# Autodesk Inventor assembly: Dog Feeder _Caja
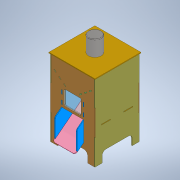
[picture p0: Inventor's stored thumbnail of the model, 180x180]
Saved by Autodesk Inventor 2020.1 (Build 241239000, 239)
## iProperties
Created: 2019-12-08
Part Number: Dog Feeder _Caja
Document SubType Name: Assembly
Designer: Daniel
Author: Daniel
## Documents named in this file (18)
- F:\Proyectos\Dog Feeder\Solido\Version Caja\Dog Feeder _Caja.iam
- F:\Proyectos\Dog Feeder\Solido\Ensamble Inicial\Ensamble inicial_ Dog Feeder.iam
- F:\Proyectos\Dog Feeder\Solido\Version Caja\Soporte_Rodamientos.ipt
- F:\Proyectos\Dog Feeder\Solido\Version Caja\Soporte2_Rodamientos.ipt
- F:\Proyectos\Dog Feeder\Solido\Rodamiento\6202-Z.iam
- F:\Proyectos\Dog Feeder\Solido\Version Caja\Rampa.ipt
- F:\Proyectos\Dog Feeder\Solido\Version Caja\Suelo.ipt
- F:\Proyectos\Dog Feeder\Solido\Version Caja\Pared_Lateral.ipt
- F:\Proyectos\Dog Feeder\Solido\Version Caja\Pared_Trasera.ipt
- F:\Proyectos\Dog Feeder\Solido\Version Caja\Tolva_Largo.ipt
- F:\Proyectos\Dog Feeder\Solido\Version Caja\Tolva_Corto.ipt
- F:\Proyectos\Dog Feeder\Solido\Version Caja\Pared_Frontal.ipt
- F:\Proyectos\Dog Feeder\Solido\Version Caja\Ventana.ipt
- F:\Proyectos\Dog Feeder\Solido\Circuito Electrico\Circuito_Electrico.iam
- F:\Proyectos\Dog Feeder\Solido\Version Caja\Pared_Lateral_ConCircuito.ipt
- F:\Proyectos\Dog Feeder\Solido\Version Caja\Soporte_Plug_Alimentacion.ipt
- F:\Proyectos\Dog Feeder\Solido\Version Caja\Tapa.ipt
- F:\Proyectos\Dog Feeder\Solido\Removedor\Removedor.iam
## Components (22 placed, 17 different names)
1. Ensamble inicial_ Dog Feeder:1 [sub-assembly] — Insert:1, Insert:2, Insert:7, Rotational:1, Rotational:2, Flush:7, Tangent:1
2. 6202-Z:2 [sub-assembly] — Rotational:2
3. Soporte2_Rodamientos:1 — Insert:3, Insert:4
4. Soporte_Rodamientos:1 — Flush:1, Insert:1, Insert:2, Insert:3, Insert:4, Flush:2, Flush:10
5. 6202-Z:1 [sub-assembly] — Rotational:1
6. Rampa:1 — Rigid:1
7. Soporte2_Rodamientos:2 — Insert:6
8. Soporte_Rodamientos:2 — Insert:6, Insert:7, Flush:2, Flush:3, Mate:1, Mate:2, Rigid:1
9. Suelo:1 — Flush:3, Mate:1, Mate:2, Flush:4, Rigid:2, Flush:5, Rigid:4, Mate:12
10. Tolva_Corto:1 — Flush:7, Mate:4, Mate:5, Flush:9
11. Tolva_Corto:2 — Flush:9, Mate:6, Mate:7
12. Tolva_Largo:1 — Flush:6, Rigid:5, Mate:4, Mate:5, Mate:6
13. Tolva_Largo:2 — Rigid:3, Mate:7
14. Pared_Trasera:1 — Flush:5, Flush:6, Rigid:3, Flush:8, Rigid:5, Mate:9, Flush:15, Flush:16
15. Pared_Lateral:1 — Flush:4, Rigid:4
16. Pared_Lateral_ConCircuito:1 — Rigid:2, Flush:8, Mate:9, Flush:11, Flush:12, Mate:10, Mate:11, Flush:14, Flush:18
17. Pared_Frontal:1 — Flush:10, Flush:11, Flush:12, Flush:13, Flush:17, Mate:13
18. Ventana:1 — Flush:13
19. Circuito_Electrico:1 [sub-assembly] — Mate:10, Mate:11, Flush:14
20. Soporte_Plug_Alimentacion:1 — Flush:15, Mate:12, Flush:16
21. Tapa:1 — Flush:17, Mate:13, Flush:18, Cylindrical:1
22. Removedor:1 [sub-assembly] — Cylindrical:1, Tangent:1
## Relationships (44: Flush 18, Mate 11, Insert 6, WeldJoint 5, RevoluteJoint 2, CylindricalJoint 1, Tangent 1)
- Flush:1 (-59.46 mm): Soporte_Rodamientos:1
- Insert:1: Ensamble inicial_ Dog Feeder:1 ↔ Soporte_Rodamientos:1
- Insert:2: Ensamble inicial_ Dog Feeder:1 ↔ Soporte_Rodamientos:1
- Insert:3: Soporte2_Rodamientos:1 ↔ Soporte_Rodamientos:1
- Insert:4: Soporte2_Rodamientos:1 ↔ Soporte_Rodamientos:1
- Insert:6: Soporte2_Rodamientos:2 ↔ Soporte_Rodamientos:2
- Insert:7: Ensamble inicial_ Dog Feeder:1 ↔ Soporte_Rodamientos:2
- Flush:2: Soporte_Rodamientos:1 ↔ Soporte_Rodamientos:2
- Rotational:1 [RevoluteJoint]: Ensamble inicial_ Dog Feeder:1 ↔ 6202-Z:1
- Rotational:2 [RevoluteJoint]: Ensamble inicial_ Dog Feeder:1 ↔ 6202-Z:2
- Flush:3: Soporte_Rodamientos:2 ↔ Suelo:1
- Mate:1: Soporte_Rodamientos:2 ↔ Suelo:1
- Mate:2: Soporte_Rodamientos:2 ↔ Suelo:1
- Rigid:1 [WeldJoint]: Rampa:1 ↔ Soporte_Rodamientos:2
- Flush:4: Suelo:1 ↔ Pared_Lateral:1
- Rigid:2 [WeldJoint]: Suelo:1 ↔ Pared_Lateral_ConCircuito:1
- Flush:5: Suelo:1 ↔ Pared_Trasera:1
- Flush:6: Tolva_Largo:1 ↔ Pared_Trasera:1
- Flush:7: Ensamble inicial_ Dog Feeder:1 ↔ Tolva_Corto:1
- Rigid:3 [WeldJoint]: Tolva_Largo:2 ↔ Pared_Trasera:1
- Rigid:4 [WeldJoint]: Suelo:1 ↔ Pared_Lateral:1
- Flush:8: Pared_Trasera:1 ↔ Pared_Lateral_ConCircuito:1
- Rigid:5 [WeldJoint]: Tolva_Largo:1 ↔ Pared_Trasera:1
- Mate:4: Tolva_Corto:1 ↔ Tolva_Largo:1
- Mate:5: Tolva_Corto:1 ↔ Tolva_Largo:1
- Flush:9: Tolva_Corto:1 ↔ Tolva_Corto:2
- Mate:6: Tolva_Corto:2 ↔ Tolva_Largo:1
- Mate:7: Tolva_Corto:2 ↔ Tolva_Largo:2
- Flush:10: Soporte_Rodamientos:1 ↔ Pared_Frontal:1
- Mate:9: Pared_Trasera:1 ↔ Pared_Lateral_ConCircuito:1
- Flush:11: Pared_Lateral_ConCircuito:1 ↔ Pared_Frontal:1
- Flush:12: Pared_Lateral_ConCircuito:1 ↔ Pared_Frontal:1
- Flush:13: Pared_Frontal:1 ↔ Ventana:1
- Mate:10: Pared_Lateral_ConCircuito:1 ↔ Circuito_Electrico:1
- Mate:11: Pared_Lateral_ConCircuito:1 ↔ Circuito_Electrico:1
- Flush:14 (73 mm): Pared_Lateral_ConCircuito:1 ↔ Circuito_Electrico:1
- Flush:15: Pared_Trasera:1 ↔ Soporte_Plug_Alimentacion:1
- Mate:12 (20 mm): Suelo:1 ↔ Soporte_Plug_Alimentacion:1
- Flush:16 (5 mm): Pared_Trasera:1 ↔ Soporte_Plug_Alimentacion:1
- Flush:17 (3 mm): Pared_Frontal:1 ↔ Tapa:1
- Mate:13: Pared_Frontal:1 ↔ Tapa:1
- Flush:18 (3 mm): Pared_Lateral_ConCircuito:1 ↔ Tapa:1
- Cylindrical:1: Tapa:1 ↔ Removedor:1
- Tangent:1 (1 mm): Ensamble inicial_ Dog Feeder:1 ↔ Removedor:1
